# Autodesk Inventor assembly: Ring Stand
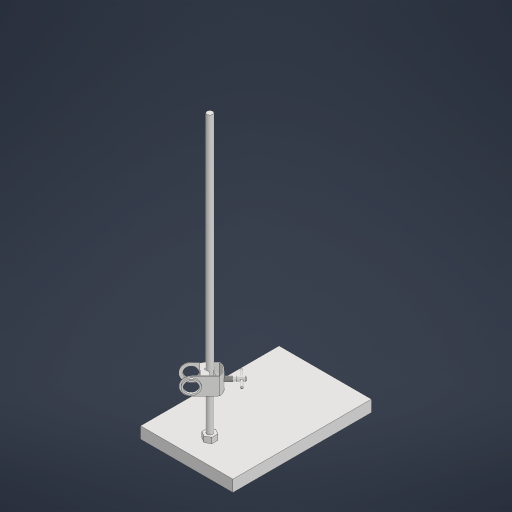
[picture p0: Inventor's stored thumbnail of the model, 512x512]
Saved by Autodesk Inventor 2023.1 (Build 271208000, 208)
## iProperties
Created: 2022-12-06
Part Number: Ring Stand
Document SubType Name: Assembly
Designer: aubrey-work
Author: aubrey-work
## Documents named in this file (4)
- C:\GitHubRepos\PHYS-12-Website\content\portfolio\FRC Floor Layout\Aubreys\Graduated Shelves\Ring Stand.iam
- C:\GitHubRepos\PHYS-12-Website\content\portfolio\FRC Floor Layout\Aubreys\Graduated Shelves\Ring Stand.ipt
- C:\GitHubRepos\PHYS-12-Website\content\portfolio\FRC Floor Layout\Aubreys\Graduated Shelves\Clamp Body.ipt
- C:\GitHubRepos\PHYS-12-Website\content\portfolio\FRC Floor Layout\Aubreys\Graduated Shelves\Clamp Screw.ipt
## Components (3 placed, 3 different names)
1. Ring Stand:1 — Mate:2, Mate:3
2. Clamp Body:1 — Mate:1, Mate:2
3. Clamp Screw:1 — Mate:1, Mate:3
## Relationships (3: Mate 3)
- Mate:1: Clamp Body:1 ↔ Clamp Screw:1
- Mate:2: Ring Stand:1 ↔ Clamp Body:1
- Mate:3 (6.35 mm): Ring Stand:1 ↔ Clamp Screw:1
